# Autodesk Inventor assembly: MIRカウンター展開システム
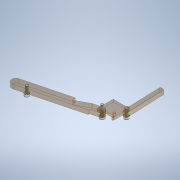
[picture p0: Inventor's stored thumbnail of the model, 180x180]
Saved by Autodesk Inventor 2020.2 (Build 242310000, 310)
## iProperties
Created: 2020-04-03
Part Number: MIRカウンター展開システム
Document SubType Name: Assembly
Designer: aoyama
Mass: 8.99488 g
Surface Area: 55.3605 cm^2
Volume: 6.96361 cm^3
Density: 1.2917 g/cm^3
Author: aoyama
## Documents named in this file (6)
- C:\Users\aoyam\Desktop\SRDC_local\Inventor\二年機\インナー4層丙参型\全体\MIR達\MIRカウンター展開システム.iam
- C:\Users\aoyam\Desktop\SRDC_local\Inventor\二年機\インナー4層丙参型\全体\MIR達\MIRカウンター.ipt
- C:\Users\aoyam\Desktop\SRDC_local\Inventor\二年機\インナー4層丙参型\全体\MIR達\MIRカウンター展開.ipt
- C:\Users\aoyam\Desktop\SRDC_local\Inventor\二年機\インナー4層丙参型\全体\MIR達\MIRカウンター展開支柱test.ipt
- C:\Users\aoyam\Desktop\SRDC_local\Inventor\二年機\インナー4層丙参型\汎用部品\ネジアルミM3L12.ipt
- C:\Users\aoyam\Desktop\SRDC_local\Inventor\二年機\インナー4層丙参型\汎用部品\ネジアルミM3L8.ipt
## Components (6 placed, 5 different names)
1. MIRカウンター:1 — 挿入:10, 挿入:12, 挿入:13
2. MIRカウンター展開:1 — 挿入:9, 挿入:11
3. MIRカウンター展開支柱test:1 — 挿入:9, 挿入:13
4. ネジアルミM3L12:1 — 挿入:10
5. ネジアルミM3L8:1 — 挿入:11
6. ネジアルミM3L8:2 — 挿入:12
## Relationships (5: Insert 5)
- 挿入:9 [Insert]: MIRカウンター展開:1 ↔ MIRカウンター展開支柱test:1
- 挿入:10 [Insert]: MIRカウンター:1 ↔ ネジアルミM3L12:1
- 挿入:11 [Insert]: MIRカウンター展開:1 ↔ ネジアルミM3L8:1
- 挿入:12 [Insert] (3 mm): MIRカウンター:1 ↔ ネジアルミM3L8:2
- 挿入:13 [Insert]: MIRカウンター:1 ↔ MIRカウンター展開支柱test:1
